# Autodesk Inventor assembly: battery for holder
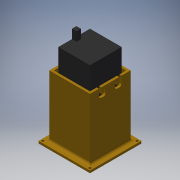
[picture p0: Inventor's stored thumbnail of the model, 180x180]
Saved by Autodesk Inventor 2017 (Build 210142000, 142)
## iProperties
Created: 2018-01-10
Part Number: battery for holder
Document SubType Name: Assembly
Designer: User
Author: User
## Documents named in this file (3)
- C:\Robotics\CAD\2017-18_CAD\battery for holder.iam
- C:\Robotics\CAD\2017-18_CAD\bateryHolder2.0.ipt
- C:\Robotics\CAD\2017-18_CAD\batery.ipt
## Components (2 placed, 2 different names)
1. bateryHolder2..0:1 — Mate:1, Mate:2, Mate:3
2. batery:1 — Mate:1, Mate:2, Mate:3
## Relationships (3: Mate 3)
- Mate:1 (3.175 mm): bateryHolder2..0:1 ↔ batery:1
- Mate:2 (3.175 mm): bateryHolder2..0:1 ↔ batery:1
- Mate:3: bateryHolder2..0:1 ↔ batery:1
